# Autodesk Inventor assembly: CT3x3
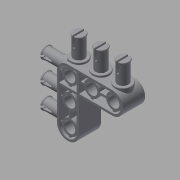
[picture p0: Inventor's stored thumbnail of the model, 180x180]
Saved by Autodesk Inventor 2019.3 (Build 233278000, 278)
## iProperties
Created: 2019-01-31
Part Number: CT3x3
Document SubType Name: Assembly
Designer: Varga Daniel
Vertical_hole_count: 3,000 ul
Horizontal_hole_count: 3,000 ul
Author: Varga Daniel
## Documents named in this file (10)
- C:\!_Dani\!_cloud\OneDrive\!_munka\Revolution\RevvyDemoKit\Structural parts\Connector Boxes\Connector triangle\CT2+x2+.iam
- C:\!_Dani\!_cloud\OneDrive\!_munka\Revolution\RevvyDemoKit\Structural parts\Beams\beam_single_end_part.ipt
- C:\!_Dani\!_cloud\OneDrive\!_munka\Revolution\RevvyDemoKit\Structural parts\Beams\beam_single_inner_part.ipt
- C:\!_Dani\!_cloud\OneDrive\!_munka\Revolution\RevvyDemoKit\Structural parts\Connetor Pins\Connector_pin_stick.ipt
- C:\!_Dani\!_cloud\OneDrive\!_munka\Revolution\RevvyDemoKit\Structural parts\Connector Boxes\Connector_box_collar\Connector_box_collar-one_side.ipt
- C:\!_Dani\!_cloud\OneDrive\!_munka\Revolution\RevvyDemoKit\Structural parts\Connector Boxes\Connector_box_collar.ipt
- C:\!_Dani\!_cloud\OneDrive\!_munka\Revolution\RevvyDemoKit\Structural parts\Connector Boxes\Connector triangle\Connector_triangle_L_base.ipt
- C:\!_Dani\!_cloud\OneDrive\!_munka\Revolution\RevvyDemoKit\Structural parts\Connector Boxes\Connector_box_collar\Connector_box_collar-None.ipt
- CT2x2.iam
- CT3x3.iam
## Components (17 placed, 6 different names)
1. Connector_triangle_L_base:1 — Mate:40, Mate:41, Angle:5, Mate:42, Mate:43, Angle:6, Flush:1, Flush:2, Mate:46, Flush:3, Flush:4, Mate:49, Flush:5, Mate:50, Flush:6, Flush:7, Flush:8, Mate:55
2. beam_single_end_part:1 — Mate:37, Mate:38, Mate:39, Angle:4, Flush:7, Flush:8, Mate:55
3. beam_single_end_part:2 — Mate:28, Mate:29, Angle:1, Mate:36, Flush:3, Flush:4, Mate:49
4. Connector_box_collar-one_side:1 — Mate:18, Mate:19, Mate:37, Mate:38
5. Connector_pin_stick:2 — Mate:18, Mate:19, Mate:39, Angle:4
6. Connector_box_collar-one_side:3 — Mate:41
7. Connector_pin_stick:3 — Mate:40, Angle:5
8. Connector_box_collar-one_side:4 — Mate:43
9. Connector_pin_stick:4 — Mate:42, Angle:6
10. Connector_box_collar-one_side:5 — Mate:28, Mate:29
11. Connector_pin_stick:5 — Angle:1, Mate:36
12. Connector_box_collar-None:6 — Mate:48
13. Connector_box_collar-None:7 — Mate:53
14. beam_single_inner_part:2 — Flush:5, Mate:50, Flush:6, Mate:53, Mate:54, Angle:8
15. Connector_pin_stick:7 — Mate:54, Angle:8
16. beam_single_inner_part:3 — Flush:1, Flush:2, Mate:46, Mate:47, Mate:48, Angle:7
17. Connector_pin_stick:6 — Mate:47, Angle:7
## Component patterns: (1 elements, first: beam_single_inner_part:2 + Connector_pin_stick:7), (1 elements, first: beam_single_inner_part:3 + Connector_pin_stick:6)
## Relationships (44: Mate 30, Flush 8, Angle 6)
- Mate:18: Connector_box_collar-one_side:1 ↔ Connector_pin_stick:2
- Mate:19: Connector_box_collar-one_side:1 ↔ Connector_pin_stick:2
- [Mate]: Connector_box_collar-one_side:3 ↔ Connector_pin_stick:3
- [Mate]: Connector_box_collar-one_side:3 ↔ Connector_pin_stick:3
- [Mate]: Connector_box_collar-one_side:4 ↔ Connector_pin_stick:4
- [Mate]: Connector_box_collar-one_side:4 ↔ Connector_pin_stick:4
- [Mate]: Connector_box_collar-one_side:5 ↔ Connector_pin_stick:5
- [Mate]: Connector_box_collar-one_side:5 ↔ Connector_pin_stick:5
- Mate:28: beam_single_end_part:2 ↔ Connector_box_collar-one_side:5
- Mate:29: beam_single_end_part:2 ↔ Connector_box_collar-one_side:5
- Angle:1 (0 deg): beam_single_end_part:2 ↔ Connector_pin_stick:5
- Mate:36: beam_single_end_part:2 ↔ Connector_pin_stick:5
- Mate:37: beam_single_end_part:1 ↔ Connector_box_collar-one_side:1
- Mate:38: beam_single_end_part:1 ↔ Connector_box_collar-one_side:1
- Mate:39: beam_single_end_part:1 ↔ Connector_pin_stick:2
- Angle:4 (0 deg): beam_single_end_part:1 ↔ Connector_pin_stick:2
- Mate:40: Connector_triangle_L_base:1 ↔ Connector_pin_stick:3
- Mate:41: Connector_triangle_L_base:1 ↔ Connector_box_collar-one_side:3
- Angle:5 (0 deg): Connector_triangle_L_base:1 ↔ Connector_pin_stick:3
- Mate:42: Connector_triangle_L_base:1 ↔ Connector_pin_stick:4
- Mate:43: Connector_triangle_L_base:1 ↔ Connector_box_collar-one_side:4
- Angle:6 (0 deg): Connector_triangle_L_base:1 ↔ Connector_pin_stick:4
- [Mate]: Connector_box_collar-None:6 ↔ Connector_pin_stick:6
- [Mate]: Connector_box_collar-None:6 ↔ Connector_pin_stick:6
- Flush:1: Connector_triangle_L_base:1 ↔ beam_single_inner_part:3
- Flush:2: Connector_triangle_L_base:1 ↔ beam_single_inner_part:3
- Mate:46: Connector_triangle_L_base:1 ↔ beam_single_inner_part:3
- Mate:47: beam_single_inner_part:3 ↔ Connector_pin_stick:6
- Mate:48: Connector_box_collar-None:6 ↔ beam_single_inner_part:3
- Angle:7 (0 deg): beam_single_inner_part:3 ↔ Connector_pin_stick:6
- Flush:3: Connector_triangle_L_base:1 ↔ beam_single_end_part:2
- Flush:4: Connector_triangle_L_base:1 ↔ beam_single_end_part:2
- Mate:49 (10 mm): Connector_triangle_L_base:1 ↔ beam_single_end_part:2
- Flush:5: Connector_triangle_L_base:1 ↔ beam_single_inner_part:2
- Mate:50: Connector_triangle_L_base:1 ↔ beam_single_inner_part:2
- Flush:6: Connector_triangle_L_base:1 ↔ beam_single_inner_part:2
- [Mate]: Connector_box_collar-None:7 ↔ Connector_pin_stick:7
- [Mate]: Connector_box_collar-None:7 ↔ Connector_pin_stick:7
- Mate:53: Connector_box_collar-None:7 ↔ beam_single_inner_part:2
- Mate:54: beam_single_inner_part:2 ↔ Connector_pin_stick:7
- Angle:8 (0 deg): beam_single_inner_part:2 ↔ Connector_pin_stick:7
- Flush:7: Connector_triangle_L_base:1 ↔ beam_single_end_part:1
- Flush:8: Connector_triangle_L_base:1 ↔ beam_single_end_part:1
- Mate:55 (10 mm): Connector_triangle_L_base:1 ↔ beam_single_end_part:1
## Named parameters: Vertical_hole_count = 3, Horizontal_hole_count = 3, d53_d49 = 0 mm, d54_d50 = 0 mm, d55_d49 = 0 mm, d56_d50 = 0 mm, d57_d49 = 0 mm, d58_d50 = 0 mm, d97_d55_d49 = 0 mm, d98_d56_d50 = 0 mm, d111_d97_d55_d49 = 0 mm, d112_d98_d56_d50 = 0 mm
